# Autodesk Inventor assembly: Jetson & Carrier Board
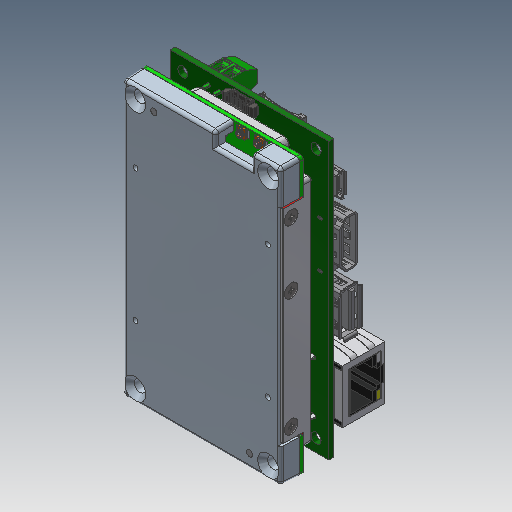
[picture p0: Inventor's stored thumbnail of the model, 512x512]
Saved by Autodesk Inventor 2019.4 (Build 234330000, 330)
## iProperties
Created: 2019-07-17
Part Number: Jetson & Carrier Board
Material: 一般
Document SubType Name: Assembly
Designer: y6tada
Author: y6tada
## Documents named in this file (3)
- C:\Workspace\Yuni9\Inventor\Libs\Jetson & Carrier Board\Jetson & Carrier Board.iam
- C:\Workspace\Yuni9\Inventor\Libs\Jetson & Carrier Board\Jetson TX2\jetson_tx2_with_housing.iam
- C:\Workspace\Yuni9\Inventor\Libs\Jetson & Carrier Board\ASG003\ASG003.iam
## Components (2 placed, 2 different names)
1. jetson_tx2_with_housing:1 [sub-assembly] — メイト:1, フラッシュ:1, メイト:6, メイト:7, メイト:8
2. ASG003:1 [sub-assembly] — メイト:5, メイト:6, メイト:7, メイト:8
## Relationships (6: Mate 5, Flush 1)
- メイト:1 [Mate]: jetson_tx2_with_housing:1
- フラッシュ:1 [Flush]: jetson_tx2_with_housing:1
- メイト:5 [Mate]: ASG003:1
- メイト:6 [Mate]: jetson_tx2_with_housing:1 ↔ ASG003:1
- メイト:7 [Mate]: jetson_tx2_with_housing:1 ↔ ASG003:1
- メイト:8 [Mate] (8 mm): jetson_tx2_with_housing:1 ↔ ASG003:1
